# Autodesk Inventor assembly: Assembly1
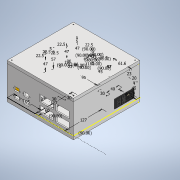
[picture p0: Inventor's stored thumbnail of the model, 180x180]
Saved by Autodesk Inventor 2020.2 (Build 242310000, 310)
## iProperties
Created: 2020-01-31
Part Number: Assembly1
Document SubType Name: Assembly
Designer: ColinP
Author: ColinP
## Documents named in this file (8)
- C:\Users\ColinP\Documents\Inventor\HeaterControlIQC\Assembly1.iam
- C:\Users\ColinP\Documents\Inventor\HeaterControlIQC\bakeoutbox.ipt
- C:\Users\ColinP\Documents\Inventor\HeaterControlIQC\User Library-Thermocouple_Submini Jack.ipt
- C:\Users\ColinP\Documents\Inventor\HeaterControlIQC\Qualtek_06AE2.ipt
- C:\Users\ColinP\Documents\Inventor\HeaterControlIQC\4300-0705.ipt
- C:\Users\ColinP\Documents\Inventor\HeaterControlIQC\CUI_VSK-S5-5UA-T (1)\CUI_VSK-S5-5UA-T.iam
- C:\Users\ColinP\Documents\Inventor\HeaterControlIQC\OnShore_ES100006DS.ipt
- C:\Users\ColinP\Documents\Inventor\HeaterControlIQC\bakeoutbox lid.ipt
## Components (14 placed, 7 different names)
1. bakeoutbox:1 — Mate:3, Flush:1, Flush:2, Flush:3, Flush:4, Flush:5, Flush:6, Flush:7, Flush:8, Flush:9, Mate:7, Mate:9, Mate:10, Mate:11, Mate:12, Mate:13, Mate:14, Mate:15, Mate:16, Mate:17, Mate:18, Mate:19, Mate:20, Mate:21, Mate:22, Mate:23, Mate:24, Mate:27, Mate:28, Mate:29, Mate:30, Mate:31, Mate:32, Mate:33, Mate:34, Mate:35, Mate:36, Mate:37, Mate:38
2. User Library-Thermocouple_Submini Jack:1 — Mate:16, Mate:17, Mate:18
3. User Library-Thermocouple_Submini Jack:2 — Mate:7, Mate:9, Mate:19
4. User Library-Thermocouple_Submini Jack:3 — Mate:10, Mate:11, Mate:12
5. User Library-Thermocouple_Submini Jack:4 — Mate:13, Mate:14, Mate:15
6. Qualtek_06AE2:1 — Mate:3, Mate:20, Mate:21
7. 4300-0705:1 — Flush:7, Flush:8, Flush:9
8. 4300-0705:2 — Flush:4, Flush:5, Flush:6
9. 4300-0705:3 — Flush:1, Flush:2, Flush:3
10. CUI_VSK-S5-5UA-T:1 [sub-assembly] — Mate:22, Mate:23, Mate:24
11. OnShore_ES100006DS:1 — Mate:27, Mate:34, Mate:35
12. OnShore_ES100006DS:2 — Mate:28, Mate:29, Mate:30
13. OnShore_ES100006DS:3 — Mate:31, Mate:32, Mate:33
14. bakeoutbox lid:1 — Mate:36, Mate:37, Mate:38
## Relationships (39: Mate 30, Flush 9)
- Mate:3: bakeoutbox:1 ↔ Qualtek_06AE2:1
- Flush:1: bakeoutbox:1 ↔ 4300-0705:3
- Flush:2: bakeoutbox:1 ↔ 4300-0705:3
- Flush:3: bakeoutbox:1 ↔ 4300-0705:3
- Flush:4: bakeoutbox:1 ↔ 4300-0705:2
- Flush:5: bakeoutbox:1 ↔ 4300-0705:2
- Flush:6: bakeoutbox:1 ↔ 4300-0705:2
- Flush:7: bakeoutbox:1 ↔ 4300-0705:1
- Flush:8: bakeoutbox:1 ↔ 4300-0705:1
- Flush:9: bakeoutbox:1 ↔ 4300-0705:1
- Mate:7: bakeoutbox:1 ↔ User Library-Thermocouple_Submini Jack:2
- Mate:9: bakeoutbox:1 ↔ User Library-Thermocouple_Submini Jack:2
- Mate:10: bakeoutbox:1 ↔ User Library-Thermocouple_Submini Jack:3
- Mate:11: bakeoutbox:1 ↔ User Library-Thermocouple_Submini Jack:3
- Mate:12: bakeoutbox:1 ↔ User Library-Thermocouple_Submini Jack:3
- Mate:13: bakeoutbox:1 ↔ User Library-Thermocouple_Submini Jack:4
- Mate:14: bakeoutbox:1 ↔ User Library-Thermocouple_Submini Jack:4
- Mate:15: bakeoutbox:1 ↔ User Library-Thermocouple_Submini Jack:4
- Mate:16: bakeoutbox:1 ↔ User Library-Thermocouple_Submini Jack:1
- Mate:17: bakeoutbox:1 ↔ User Library-Thermocouple_Submini Jack:1
- Mate:18: bakeoutbox:1 ↔ User Library-Thermocouple_Submini Jack:1
- Mate:19: bakeoutbox:1 ↔ User Library-Thermocouple_Submini Jack:2
- Mate:20: bakeoutbox:1 ↔ Qualtek_06AE2:1
- Mate:21: bakeoutbox:1 ↔ Qualtek_06AE2:1
- Mate:22: bakeoutbox:1 ↔ CUI_VSK-S5-5UA-T:1
- Mate:23: bakeoutbox:1 ↔ CUI_VSK-S5-5UA-T:1
- Mate:24: bakeoutbox:1 ↔ CUI_VSK-S5-5UA-T:1
- Mate:27: bakeoutbox:1 ↔ OnShore_ES100006DS:1
- Mate:28: bakeoutbox:1 ↔ OnShore_ES100006DS:2
- Mate:29: bakeoutbox:1 ↔ OnShore_ES100006DS:2
- Mate:30: bakeoutbox:1 ↔ OnShore_ES100006DS:2
- Mate:31: bakeoutbox:1 ↔ OnShore_ES100006DS:3
- Mate:32: bakeoutbox:1 ↔ OnShore_ES100006DS:3
- Mate:33: bakeoutbox:1 ↔ OnShore_ES100006DS:3
- Mate:34: bakeoutbox:1 ↔ OnShore_ES100006DS:1
- Mate:35: bakeoutbox:1 ↔ OnShore_ES100006DS:1
- Mate:36: bakeoutbox:1 ↔ bakeoutbox lid:1
- Mate:37: bakeoutbox:1 ↔ bakeoutbox lid:1
- Mate:38: bakeoutbox:1 ↔ bakeoutbox lid:1
